# Autodesk Inventor assembly: holder 1
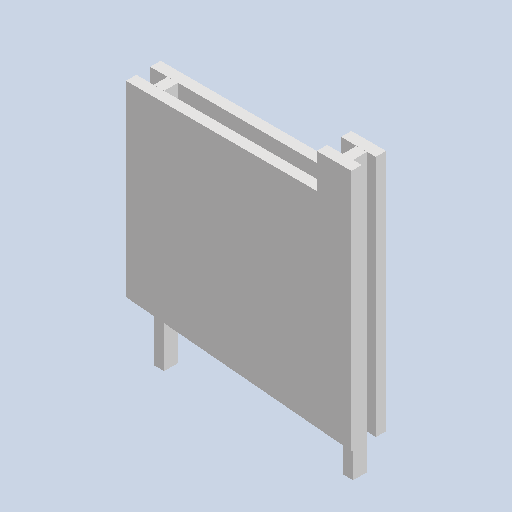
[picture p0: Inventor's stored thumbnail of the model, 512x512]
Saved by Autodesk Inventor 2025.3 (Build 293356000, 356)
## iProperties
Created: 2026-04-27
Part Number: holder 1
Document SubType Name: Assembly
Designer: kamal
Author: kamal
## Documents named in this file (4)
- C:\Users\kamal\OneDrive\Desktop\Personal\semester 4\Basics of Mechatronics\Full Assembly\holder 1.iam
- C:\Users\kamal\OneDrive\Desktop\Personal\semester 4\Basics of Mechatronics\Full Assembly\support select pt 1.ipt
- C:\Users\kamal\OneDrive\Desktop\Personal\semester 4\Basics of Mechatronics\Full Assembly\select holder pt 2.ipt
- C:\Users\kamal\OneDrive\Desktop\Personal\semester 4\Basics of Mechatronics\Full Assembly\select holder pt 3.ipt
## Components (4 placed, 3 different names)
1. support select pt 1:1 — Mate:3, Mate:4, Mate:5
2. support select pt 1:2 — Mate:3, Mate:6, Mate:7, Mate:8, Mate:9
3. select holder pt 2:1 — Mate:4, Mate:5, Mate:6, Mate:7
4. select holder pt 3:1 — Mate:8, Mate:9
## Relationships (7: Mate 7)
- Mate:3 (4 mm): support select pt 1:1 ↔ support select pt 1:2
- Mate:4: support select pt 1:1 ↔ select holder pt 2:1
- Mate:5: support select pt 1:1 ↔ select holder pt 2:1
- Mate:6: support select pt 1:2 ↔ select holder pt 2:1
- Mate:7: support select pt 1:2 ↔ select holder pt 2:1
- Mate:8: support select pt 1:2 ↔ select holder pt 3:1
- Mate:9: support select pt 1:2 ↔ select holder pt 3:1
